# Autodesk Inventor assembly: Skateboard Remote
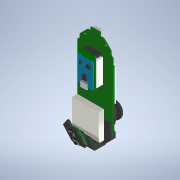
[picture p0: Inventor's stored thumbnail of the model, 180x180]
Saved by Autodesk Inventor 2020 (Build 240168000, 168)
## iProperties
Created: 2021-01-14
Part Number: Skateboard Remote
Document SubType Name: Assembly
Designer: Luke
Author: Luke
## Documents named in this file (14)
- C:\Users\Luke\Documents\Git Projects\Electric Skateboard V2\Part Files\Remote Parts\Skateboard Remote.iam
- C:\Users\Luke\Documents\Git Projects\Electric Skateboard V2\Part Files\Remote Parts\PCB.ipt
- C:\Users\Luke\Documents\Git Projects\Electric Skateboard V2\Part Files\Remote Parts\Battery Spacer.ipt
- C:\Users\Luke\Documents\Git Projects\Electric Skateboard V2\Part Files\Remote Parts\Battery.ipt
- C:\Users\Luke\Documents\Git Projects\Electric Skateboard V2\Part Files\Remote Parts\Button Module.ipt
- C:\Users\Luke\Documents\Git Projects\Electric Skateboard V2\Part Files\Remote Parts\Joystick.ipt
- C:\Users\Luke\Documents\Git Projects\Electric Skateboard V2\Part Files\Remote Parts\Button.ipt
- C:\Users\Luke\Documents\Git Projects\Electric Skateboard V2\Part Files\Remote Parts\Button Holder Top.ipt
- C:\Users\Luke\Documents\Git Projects\Electric Skateboard V2\Part Files\Remote Parts\Button Holder Bottom Newest Angle.ipt
- C:\Users\Luke\Documents\Git Projects\Electric Skateboard V2\Part Files\Remote Parts\Joystick Cap.ipt
- C:\Users\Luke\Documents\Git Projects\Electric Skateboard V2\Part Files\Remote Parts\Display.ipt
- C:\Users\Luke\Documents\Git Projects\Electric Skateboard V2\Part Files\Remote Parts\Vibrator Motor.ipt
- C:\Users\Luke\Documents\Git Projects\Electric Skateboard V2\Part Files\Remote Parts\USB Port.ipt
- C:\Users\Luke\Documents\Git Projects\Electric Skateboard V2\Part Files\Remote Parts\BMS.ipt
## Components (15 placed, 13 different names)
1. PCB:1 — Mate:1, Flush:1, Flush:2, Mate:2, Flush:6, Flush:8, Flush:9, Flush:10, Mate:14, Mate:15, Mate:16, Flush:12, Mate:23, Mate:24, Mate:25, Mate:27, Mate:28, Mate:29, Mate:30, Flush:15, Mate:31, Mate:32, Flush:16
2. Battery Spacer:1 — Mate:1, Flush:1, Flush:2, Flush:3
3. Battery:1 — Flush:3, Mate:2, Flush:12
4. Button Module:1 — Mate:6, Mate:7, Mate:8, Mate:9, Mate:10, Mate:11, Mate:19, Mate:20, Flush:14
5. Joystick:1 — Flush:6, Flush:8, Flush:9, Flush:10, Mate:21, Mate:22, Mate:26
6. Button:2 — Mate:6, Mate:7, Mate:8
7. Button:3 — Mate:9, Mate:10, Mate:11
8. Button Holder Top:1 — Mate:14, Mate:15, Mate:16, Mate:17, Mate:18, Flush:13
9. Button Holder Bottom Newest Angle:1 — Mate:17, Mate:18, Flush:13, Mate:19, Mate:20, Flush:14
10. Joystick Cap:1 — Mate:21, Mate:22
11. Display:1 — Mate:23, Mate:24, Mate:25, Mate:26
12. Vibrator Motor:1 — Mate:27, Mate:28, Mate:29
13. USB Port:1 — Mate:30, Flush:15, Mate:31
14. BMS:1 — Mate:32, Flush:16, Mate:33, Flush:17, Mate:34
15. USB Port:2 — Mate:33, Flush:17, Mate:34
## Relationships (42: Mate 29, Flush 13)
- Mate:1: PCB:1 ↔ Battery Spacer:1
- Flush:1 (9.27 mm): PCB:1 ↔ Battery Spacer:1
- Flush:2 (6.4 mm): PCB:1 ↔ Battery Spacer:1
- Flush:3: Battery Spacer:1 ↔ Battery:1
- Mate:2: PCB:1 ↔ Battery:1
- Flush:6: PCB:1 ↔ Joystick:1
- Flush:8: PCB:1 ↔ Joystick:1
- Flush:9: PCB:1 ↔ Joystick:1
- Flush:10: PCB:1 ↔ Joystick:1
- Mate:6: Button Module:1 ↔ Button:2
- Mate:7: Button Module:1 ↔ Button:2
- Mate:8: Button Module:1 ↔ Button:2
- Mate:9: Button Module:1 ↔ Button:3
- Mate:10: Button Module:1 ↔ Button:3
- Mate:11: Button Module:1 ↔ Button:3
- Mate:14: PCB:1 ↔ Button Holder Top:1
- Mate:15: PCB:1 ↔ Button Holder Top:1
- Mate:16: PCB:1 ↔ Button Holder Top:1
- Flush:12 (4 mm): PCB:1 ↔ Battery:1
- Mate:17: Button Holder Top:1 ↔ Button Holder Bottom Newest Angle:1
- Mate:18: Button Holder Top:1 ↔ Button Holder Bottom Newest Angle:1
- Flush:13: Button Holder Top:1 ↔ Button Holder Bottom Newest Angle:1
- Mate:19: Button Module:1 ↔ Button Holder Bottom Newest Angle:1
- Mate:20: Button Module:1 ↔ Button Holder Bottom Newest Angle:1
- Flush:14: Button Module:1 ↔ Button Holder Bottom Newest Angle:1
- Mate:21: Joystick:1 ↔ Joystick Cap:1
- Mate:22: Joystick:1 ↔ Joystick Cap:1
- Mate:23: PCB:1 ↔ Display:1
- Mate:24: PCB:1 ↔ Display:1
- Mate:25: PCB:1 ↔ Display:1
- Mate:26 (5.5 mm): Joystick:1 ↔ Display:1
- Mate:27: PCB:1 ↔ Vibrator Motor:1
- Mate:28 (-12 mm): PCB:1 ↔ Vibrator Motor:1
- Mate:29 (-17 mm): PCB:1 ↔ Vibrator Motor:1
- Mate:30: PCB:1 ↔ USB Port:1
- Flush:15: PCB:1 ↔ USB Port:1
- Mate:31: PCB:1 ↔ USB Port:1
- Mate:32: PCB:1 ↔ BMS:1
- Flush:16: PCB:1 ↔ BMS:1
- Mate:33: BMS:1 ↔ USB Port:2
- Flush:17: BMS:1 ↔ USB Port:2
- Mate:34: BMS:1 ↔ USB Port:2
